# Autodesk Inventor assembly: ENSAMBLAJE AURA
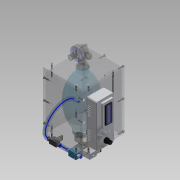
[picture p0: Inventor's stored thumbnail of the model, 180x180]
Saved by Autodesk Inventor 2019 (Build 230136000, 136)
## iProperties
Created: 2020-04-08
Part Number: ENSAMBLAJE AURA
Material: Genérico
Document SubType Name: Assembly
Designer: Luis Pujol
Author: Luis Pujol
## Documents named in this file (17)
- C:\Users\Luis Pujol\Desktop\AURA MODELADO\ENSAMBLAJE AURA.iam
- C:\Users\Luis Pujol\Desktop\AURA MODELADO\TAPA FRONTAL.ipt
- C:\Users\Luis Pujol\Desktop\AURA MODELADO\AURA RAKAN\DispositivoAura\ambu bag.ipt
- C:\Users\Luis Pujol\Desktop\AURA MODELADO\TAPA TRASERA.ipt
- C:\Users\Luis Pujol\Desktop\AURA MODELADO\TAPA INFERIOR.ipt
- C:\Users\Luis Pujol\Desktop\AURA MODELADO\TAPA SUPERIOR.ipt
- C:\Users\Luis Pujol\Desktop\AURA MODELADO\LATERAL A.ipt
- C:\Users\Luis Pujol\Desktop\AURA MODELADO\LATERAL B.ipt
- C:\Users\Luis Pujol\Documents\Inventor\Content Center Files\R2019\es-ES\ASME ANSI B18.3.5M(1)\ASME_ANSI B18.3.5M - M5x20(1).ipt
- C:\Users\Luis Pujol\Desktop\AURA MODELADO\FALSA ARANDELA.ipt
- C:\Users\Luis Pujol\Documents\Inventor\Content Center Files\R2019\es-ES\ANSI B18.3.1M(1)\ANSI B18.3.1M - M4x0,7 x 20(2).ipt
- C:\Users\Luis Pujol\Desktop\AURA MODELADO\VALVULA SELENOIDE 2V.iam
- C:\Users\Luis Pujol\Desktop\AURA MODELADO\AURA RAKAN\DispositivoAura\racor festo.ipt
- C:\Users\Luis Pujol\Desktop\AURA MODELADO\AURA RAKAN\DispositivoAura\Pneumatic Ball Valve.ipt
- C:\Users\Luis Pujol\Desktop\AURA MODELADO\ELECTRONICA\AURA ELECTRONICA\ELECTRONICA AURA ENSAMBLADA.iam
- C:\Users\Luis Pujol\Desktop\AURA MODELADO\AGARRADERA.ipt
- C:\Users\Luis Pujol\Desktop\AURA MODELADO\ENSAMBLAJE AURA\AIP\Tubos y tuberías\ENSAMBLAJE AURA.Conductos de tubos y tuberías05.iam
## Components (49 placed, 16 different names)
1. TAPA FRONTAL:1 — Coincidencia:1, Nivelación:1, Nivelación:2, Coincidencia:2, Coincidencia:3, Coincidencia:5, Nivelación:9, Nivelación:10, Nivelación:15, Coincidencia:56, Coincidencia:57, Coincidencia:58, Coincidencia:59, Coincidencia:60, Coincidencia:61, Nivelación:19
2. ambu bag:1 — Coincidencia:1, Ángulo:1, Coincidencia:74
3. TAPA TRASERA:1 — Nivelación:1, Nivelación:2, Coincidencia:2, Ángulo:1, Nivelación:3, Nivelación:7, Coincidencia:6, Coincidencia:65, Coincidencia:66, Coincidencia:67, Coincidencia:68, Coincidencia:69, Coincidencia:70, Coincidencia:74, Coincidencia:78, Coincidencia:79
4. TAPA INFERIOR:1 — Nivelación:3, Coincidencia:3, Nivelación:7, Nivelación:16, Nivelación:17, Nivelación:18
5. LATERAL A:1 — Coincidencia:5, Nivelación:9, Nivelación:14, Coincidencia:62, Coincidencia:63, Coincidencia:64, Coincidencia:83
6. LATERAL B:1 — Nivelación:10, Coincidencia:6, Coincidencia:47, Nivelación:16, Coincidencia:54, Coincidencia:71, Coincidencia:72, Coincidencia:73, Coincidencia:82
7. TAPA SUPERIOR:1 — Nivelación:14, Nivelación:15, Coincidencia:47, Coincidencia:48, Coincidencia:49, Coincidencia:50, Coincidencia:51, Coincidencia:52, Coincidencia:53, Coincidencia:84
8. FALSA ARANDELA:7 — Coincidencia:50, Coincidencia:53, Insertar:6
9. FALSA ARANDELA:8 — Coincidencia:51, Coincidencia:52, Insertar:2
10. Tornillo brochado de cabeza hueca - Métrico M4x0,7 x 20:1 — Coincidencia:54, Coincidencia:55
11. Tornillo brochado de cabeza hueca - Métrico M4x0,7 x 20:2 — Insertar:1
12. Tornillo brochado de cabeza hueca - Métrico M4x0,7 x 20:3 — Insertar:2
13. Tornillo brochado de cabeza hueca - Métrico M4x0,7 x 20:4 — Insertar:3
14. Tornillo brochado de cabeza hueca - Métrico M4x0,7 x 20:5 — Insertar:4
15. Tornillo brochado de cabeza hueca - Métrico M4x0,7 x 20:6 — Insertar:5
16. Tornillo brochado de cabeza hueca - Métrico M4x0,7 x 20:7 — Insertar:6
17. Tornillo brochado de cabeza hueca - Métrico M4x0,7 x 20:8 — Insertar:7
18. Tornillos forjados de cabeza plana avellanada con hueco hexagonal - Métricos M5x20:1 — Coincidencia:56
19. Tornillos forjados de cabeza plana avellanada con hueco hexagonal - Métricos M5x20:2 — Coincidencia:57
20. Tornillos forjados de cabeza plana avellanada con hueco hexagonal - Métricos M5x20:3 — Coincidencia:58
21. Tornillos forjados de cabeza plana avellanada con hueco hexagonal - Métricos M5x20:4 — Coincidencia:59
22. Tornillos forjados de cabeza plana avellanada con hueco hexagonal - Métricos M5x20:5 — Coincidencia:60
23. Tornillos forjados de cabeza plana avellanada con hueco hexagonal - Métricos M5x20:6 — Coincidencia:61
24. Tornillos forjados de cabeza plana avellanada con hueco hexagonal - Métricos M5x20:7 — Coincidencia:62
25. Tornillos forjados de cabeza plana avellanada con hueco hexagonal - Métricos M5x20:8 — Coincidencia:63
26. Tornillos forjados de cabeza plana avellanada con hueco hexagonal - Métricos M5x20:9 — Coincidencia:64
27. Tornillos forjados de cabeza plana avellanada con hueco hexagonal - Métricos M5x20:10 — Coincidencia:65
28. Tornillos forjados de cabeza plana avellanada con hueco hexagonal - Métricos M5x20:11 — Coincidencia:66
29. Tornillos forjados de cabeza plana avellanada con hueco hexagonal - Métricos M5x20:12 — Coincidencia:67
30. Tornillos forjados de cabeza plana avellanada con hueco hexagonal - Métricos M5x20:13 — Coincidencia:68
31. Tornillos forjados de cabeza plana avellanada con hueco hexagonal - Métricos M5x20:14 — Coincidencia:69
32. Tornillos forjados de cabeza plana avellanada con hueco hexagonal - Métricos M5x20:15 — Coincidencia:70
33. Tornillos forjados de cabeza plana avellanada con hueco hexagonal - Métricos M5x20:16 — Coincidencia:71
34. Tornillos forjados de cabeza plana avellanada con hueco hexagonal - Métricos M5x20:17 — Coincidencia:72
35. Tornillos forjados de cabeza plana avellanada con hueco hexagonal - Métricos M5x20:18 — Coincidencia:73
36. Pneumatic Ball Valve:1 — Coincidencia:78, Nivelación:17
37. VALVULA SELENOIDE 2V:1 [sub-assembly] — Coincidencia:79, Nivelación:18, Coincidencia:80, Coincidencia:81
38. racor festo:1 — Coincidencia:80
39. racor festo:2 — Coincidencia:81
40. racor festo:3 — Coincidencia:82
41. ELECTRONICA AURA ENSAMBLADA:1 [sub-assembly] — Coincidencia:83
42. AGARRADERA:1 — Coincidencia:84, Coincidencia:85, Coincidencia:86
43. Conductos de tubos y tuberías 05 [sub-assembly]
44. FALSA ARANDELA:1 — Coincidencia:48, Coincidencia:49, Insertar:7
45. FALSA ARANDELA:2 — Insertar:5
46. FALSA ARANDELA:3 — Coincidencia:55
47. FALSA ARANDELA:4 — Insertar:4
48. FALSA ARANDELA:5 — Insertar:1
49. FALSA ARANDELA:6 — Insertar:3
## Component patterns: (6 elements, first: FALSA ARANDELA:1)
## Relationships (62: Mate 42, Flush 12, Insert 7, Angle 1)
- Coincidencia:1 [Mate]: TAPA FRONTAL:1 ↔ ambu bag:1
- Nivelación:1 [Flush]: TAPA FRONTAL:1 ↔ TAPA TRASERA:1
- Nivelación:2 [Flush]: TAPA FRONTAL:1 ↔ TAPA TRASERA:1
- Coincidencia:2 [Mate] (220 mm): TAPA FRONTAL:1 ↔ TAPA TRASERA:1
- Ángulo:1 [Angle] (0 deg): ambu bag:1 ↔ TAPA TRASERA:1
- Nivelación:3 [Flush]: TAPA TRASERA:1 ↔ TAPA INFERIOR:1
- Coincidencia:3 [Mate]: TAPA FRONTAL:1 ↔ TAPA INFERIOR:1
- Nivelación:7 [Flush] (10 mm): TAPA TRASERA:1 ↔ TAPA INFERIOR:1
- Coincidencia:5 [Mate]: TAPA FRONTAL:1 ↔ LATERAL A:1
- Nivelación:9 [Flush]: TAPA FRONTAL:1 ↔ LATERAL A:1
- Nivelación:10 [Flush]: TAPA FRONTAL:1 ↔ LATERAL B:1
- Coincidencia:6 [Mate]: TAPA TRASERA:1 ↔ LATERAL B:1
- Nivelación:14 [Flush]: LATERAL A:1 ↔ TAPA SUPERIOR:1
- Nivelación:15 [Flush]: TAPA FRONTAL:1 ↔ TAPA SUPERIOR:1
- Coincidencia:47 [Mate]: LATERAL B:1 ↔ TAPA SUPERIOR:1
- Nivelación:16 [Flush]: TAPA INFERIOR:1 ↔ LATERAL B:1
- Coincidencia:48 [Mate]: TAPA SUPERIOR:1 ↔ FALSA ARANDELA:1
- Coincidencia:49 [Mate]: TAPA SUPERIOR:1 ↔ FALSA ARANDELA:1
- Coincidencia:50 [Mate]: TAPA SUPERIOR:1 ↔ FALSA ARANDELA:7
- Coincidencia:51 [Mate]: TAPA SUPERIOR:1 ↔ FALSA ARANDELA:8
- Coincidencia:52 [Mate]: TAPA SUPERIOR:1 ↔ FALSA ARANDELA:8
- Coincidencia:53 [Mate]: TAPA SUPERIOR:1 ↔ FALSA ARANDELA:7
- Coincidencia:54 [Mate]: LATERAL B:1 ↔ Tornillo brochado de cabeza hueca - Métrico M4x0,7 x 20:1
- Coincidencia:55 [Mate]: Tornillo brochado de cabeza hueca - Métrico M4x0,7 x 20:1 ↔ FALSA ARANDELA:3
- Insertar:1: Tornillo brochado de cabeza hueca - Métrico M4x0,7 x 20:2 ↔ FALSA ARANDELA:5
- Insertar:2: FALSA ARANDELA:8 ↔ Tornillo brochado de cabeza hueca - Métrico M4x0,7 x 20:3
- Insertar:3: Tornillo brochado de cabeza hueca - Métrico M4x0,7 x 20:4 ↔ FALSA ARANDELA:6
- Insertar:4: Tornillo brochado de cabeza hueca - Métrico M4x0,7 x 20:5 ↔ FALSA ARANDELA:4
- Insertar:5: Tornillo brochado de cabeza hueca - Métrico M4x0,7 x 20:6 ↔ FALSA ARANDELA:2
- Insertar:6: FALSA ARANDELA:7 ↔ Tornillo brochado de cabeza hueca - Métrico M4x0,7 x 20:7
- Insertar:7: Tornillo brochado de cabeza hueca - Métrico M4x0,7 x 20:8 ↔ FALSA ARANDELA:1
- Coincidencia:56 [Mate]: TAPA FRONTAL:1 ↔ Tornillos forjados de cabeza plana avellanada con hueco hexagonal - Métricos M5x20:1
- Coincidencia:57 [Mate]: TAPA FRONTAL:1 ↔ Tornillos forjados de cabeza plana avellanada con hueco hexagonal - Métricos M5x20:2
- Coincidencia:58 [Mate]: TAPA FRONTAL:1 ↔ Tornillos forjados de cabeza plana avellanada con hueco hexagonal - Métricos M5x20:3
- Coincidencia:59 [Mate]: TAPA FRONTAL:1 ↔ Tornillos forjados de cabeza plana avellanada con hueco hexagonal - Métricos M5x20:4
- Coincidencia:60 [Mate]: TAPA FRONTAL:1 ↔ Tornillos forjados de cabeza plana avellanada con hueco hexagonal - Métricos M5x20:5
- Coincidencia:61 [Mate]: TAPA FRONTAL:1 ↔ Tornillos forjados de cabeza plana avellanada con hueco hexagonal - Métricos M5x20:6
- Coincidencia:62 [Mate]: LATERAL A:1 ↔ Tornillos forjados de cabeza plana avellanada con hueco hexagonal - Métricos M5x20:7
- Coincidencia:63 [Mate]: LATERAL A:1 ↔ Tornillos forjados de cabeza plana avellanada con hueco hexagonal - Métricos M5x20:8
- Coincidencia:64 [Mate]: LATERAL A:1 ↔ Tornillos forjados de cabeza plana avellanada con hueco hexagonal - Métricos M5x20:9
- Coincidencia:65 [Mate]: TAPA TRASERA:1 ↔ Tornillos forjados de cabeza plana avellanada con hueco hexagonal - Métricos M5x20:10
- Coincidencia:66 [Mate]: TAPA TRASERA:1 ↔ Tornillos forjados de cabeza plana avellanada con hueco hexagonal - Métricos M5x20:11
- Coincidencia:67 [Mate]: TAPA TRASERA:1 ↔ Tornillos forjados de cabeza plana avellanada con hueco hexagonal - Métricos M5x20:12
- Coincidencia:68 [Mate]: TAPA TRASERA:1 ↔ Tornillos forjados de cabeza plana avellanada con hueco hexagonal - Métricos M5x20:13
- Coincidencia:69 [Mate]: TAPA TRASERA:1 ↔ Tornillos forjados de cabeza plana avellanada con hueco hexagonal - Métricos M5x20:14
- Coincidencia:70 [Mate]: TAPA TRASERA:1 ↔ Tornillos forjados de cabeza plana avellanada con hueco hexagonal - Métricos M5x20:15
- Coincidencia:71 [Mate]: LATERAL B:1 ↔ Tornillos forjados de cabeza plana avellanada con hueco hexagonal - Métricos M5x20:16
- Coincidencia:72 [Mate]: LATERAL B:1 ↔ Tornillos forjados de cabeza plana avellanada con hueco hexagonal - Métricos M5x20:17
- Coincidencia:73 [Mate]: LATERAL B:1 ↔ Tornillos forjados de cabeza plana avellanada con hueco hexagonal - Métricos M5x20:18
- Coincidencia:74 [Mate]: ambu bag:1 ↔ TAPA TRASERA:1
- Coincidencia:78 [Mate]: TAPA TRASERA:1 ↔ Pneumatic Ball Valve:1
- Nivelación:17 [Flush]: TAPA INFERIOR:1 ↔ Pneumatic Ball Valve:1
- Coincidencia:79 [Mate]: TAPA TRASERA:1 ↔ VALVULA SELENOIDE 2V:1
- Nivelación:18 [Flush]: TAPA INFERIOR:1 ↔ VALVULA SELENOIDE 2V:1
- Coincidencia:80 [Mate]: VALVULA SELENOIDE 2V:1 ↔ racor festo:1
- Coincidencia:81 [Mate]: VALVULA SELENOIDE 2V:1 ↔ racor festo:2
- Coincidencia:82 [Mate]: LATERAL B:1 ↔ racor festo:3
- Coincidencia:83 [Mate]: LATERAL A:1 ↔ ELECTRONICA AURA ENSAMBLADA:1
- Coincidencia:84 [Mate]: TAPA SUPERIOR:1 ↔ AGARRADERA:1
- Coincidencia:85 [Mate]: AGARRADERA:1
- Nivelación:19 [Flush] (-120 mm): TAPA FRONTAL:1
- Coincidencia:86 [Mate]: AGARRADERA:1
